# Autodesk Inventor assembly: StabilizingArm
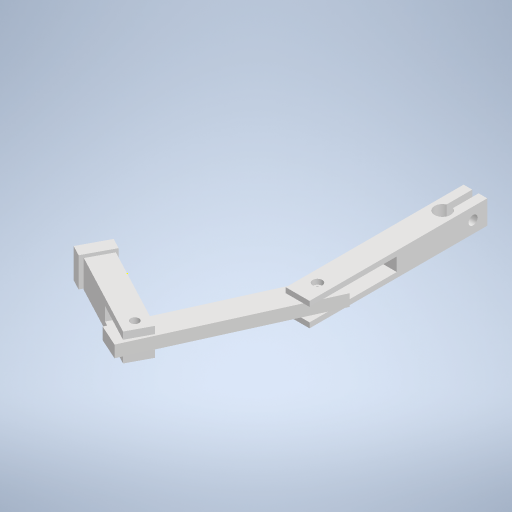
[picture p0: Inventor's stored thumbnail of the model, 512x512]
Saved by Autodesk Inventor 2024 (Build 280153000, 153)
## iProperties
Created: 2023-12-17
Part Number: StabilizingArm
Document SubType Name: Assembly
Designer: pratikhya
Author: pratikhya
## Documents named in this file (5)
- C:\Users\prati\OneDrive - IIT Kanpur\Desktop\Robot\StabilizingArm.iam
- C:\Users\prati\OneDrive - IIT Kanpur\Desktop\Robot\LInk1.ipt
- C:\Users\prati\OneDrive - IIT Kanpur\Desktop\Robot\Link2.ipt
- C:\Users\prati\OneDrive - IIT Kanpur\Desktop\Robot\Link3.ipt
- C:\Users\prati\OneDrive - IIT Kanpur\Desktop\Robot\Holder.ipt
## Components (4 placed, 4 different names)
1. LInk1:1 — Rotational:1
2. Link2:1 — Rotational:1, Rotational:4
3. Link3:1 — Rotational:3, Rotational:4
4. Holder:1 — Rotational:3
## Relationships (3: RevoluteJoint 3)
- Rotational:1 [RevoluteJoint] (1.5875 mm): LInk1:1 ↔ Link2:1
- Rotational:3 [RevoluteJoint] (2 mm): Link3:1 ↔ Holder:1
- Rotational:4 [RevoluteJoint] (-0.2 mm): Link2:1 ↔ Link3:1
